# Autodesk Inventor assembly: Assembly
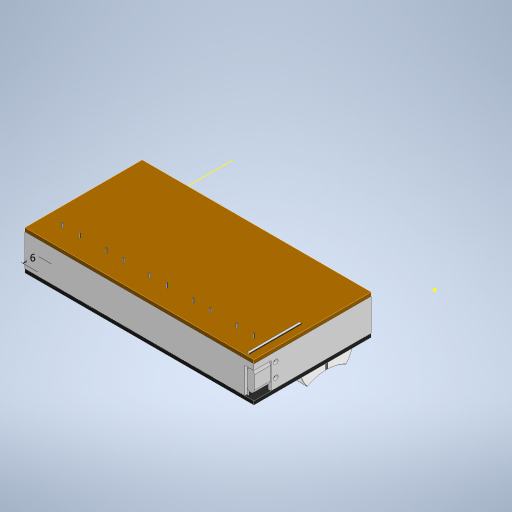
[picture p0: Inventor's stored thumbnail of the model, 512x512]
Saved by Autodesk Inventor 2023 (Build 270158000, 158)
## iProperties
Created: 2024-03-19
Part Number: Assembly
Document SubType Name: Assembly
Designer: noname
Author: noname
## Documents named in this file (10)
- C:\Users\noname\Documents\GitHub\AudMix\3dModels\Assembly.iam
- C:\Users\noname\Documents\GitHub\AudMix\3dModels\Slider\SliderAssembly.iam
- C:\Users\noname\Documents\GitHub\AudMix\3dModels\TopPCB.ipt
- C:\Users\noname\Documents\GitHub\AudMix\3dModels\Part7.ipt
- C:\Users\noname\Documents\GitHub\AudMix\3dModels\0_42_oled.ipt
- C:\Users\noname\Documents\GitHub\AudMix\3dModels\rp2040.ipt
- C:\Users\noname\Documents\GitHub\AudMix\3dModels\LedStrip\144x10.iam
- C:\Users\noname\Documents\GitHub\AudMix\3dModels\Diffuser.ipt
- C:\Users\noname\Documents\GitHub\AudMix\3dModels\Front.ipt
- C:\Users\noname\Documents\GitHub\AudMix\3dModels\Case.ipt
## Components (35 placed, 9 different names)
1. TopPCB:1 — Mate:1, Flush:1, Flush:14, Mate:9, Mate:12, Mate:16, Flush:27, Mate:17, Mate:18, Mate:19, Mate:21, Mate:23, Flush:29, Flush:32, Flush:33
2. Part7:1 — Flush:15, Mate:22, Mate:25, Flush:34, Flush:35
3. rp2040:1 — Flush:32, Flush:33
4. Front:1 — Mate:22, Mate:23, Flush:29, Mate:24
5. Case:1 — Mate:25, Flush:34, Flush:35
6. SliderAssembly:1 [sub-assembly] — Mate:1, Flush:1, Mate:11, Mate:12, Flush:30
7. 0_42_oled:5 — Flush:30, Mate:24
8. 144x10:1 [sub-assembly] — Flush:28, Mate:20, Mate:21, Flush:31
9. 144x10:2 [sub-assembly] — Mate:9, Mate:11, Mate:15, Flush:31
10. Diffuser:1 — Mate:15, Mate:16, Flush:27
11. Diffuser:2 — Mate:17, Mate:18, Mate:19, Flush:28, Mate:20
12. SliderAssembly:2 [sub-assembly]
13. 0_42_oled:6
14. 144x10:3 [sub-assembly]
15. 144x10:4 [sub-assembly]
16. Diffuser:3
17. Diffuser:4
18. SliderAssembly:3 [sub-assembly]
19. 0_42_oled:7
20. 144x10:5 [sub-assembly]
21. 144x10:6 [sub-assembly]
22. Diffuser:5
23. Diffuser:6
24. SliderAssembly:4 [sub-assembly]
25. 0_42_oled:8
26. 144x10:7 [sub-assembly]
27. 144x10:8 [sub-assembly]
28. Diffuser:7
29. Diffuser:8
30. SliderAssembly:5 [sub-assembly]
31. 0_42_oled:9
32. 144x10:9 [sub-assembly]
33. 144x10:10 [sub-assembly]
34. Diffuser:9
35. Diffuser:10
## Component patterns: (5 elements, first: SliderAssembly:1 + 0_42_oled:5 + 144x10:1 + 144x10:2 + Diffuser:1 + Diffuser:2)
## Relationships (27: Mate 15, Flush 12)
- Mate:1 (7 mm): TopPCB:1 ↔ SliderAssembly:1
- Flush:1: TopPCB:1 ↔ SliderAssembly:1
- Flush:14 (14 mm): TopPCB:1
- Flush:15: Part7:1
- Mate:9: TopPCB:1 ↔ 144x10:2
- Mate:11 (3 mm): SliderAssembly:1 ↔ 144x10:2
- Mate:12 (3.5 mm): TopPCB:1 ↔ SliderAssembly:1
- Mate:15: 144x10:2 ↔ Diffuser:1
- Mate:16: TopPCB:1 ↔ Diffuser:1
- Flush:27: TopPCB:1 ↔ Diffuser:1
- Mate:17: TopPCB:1 ↔ Diffuser:2
- Mate:18: TopPCB:1 ↔ Diffuser:2
- Mate:19: TopPCB:1 ↔ Diffuser:2
- Flush:28 (-1 mm): 144x10:1 ↔ Diffuser:2
- Mate:20: 144x10:1 ↔ Diffuser:2
- Mate:21: TopPCB:1 ↔ 144x10:1
- Mate:22: Part7:1 ↔ Front:1
- Mate:23: TopPCB:1 ↔ Front:1
- Flush:29: TopPCB:1 ↔ Front:1
- Flush:30 (3.75 mm): SliderAssembly:1 ↔ 0_42_oled:5
- Mate:24 (0.5 mm): Front:1 ↔ 0_42_oled:5
- Flush:31: 144x10:1 ↔ 144x10:2
- Flush:32 (3 mm): TopPCB:1 ↔ rp2040:1
- Flush:33 (1 mm): TopPCB:1 ↔ rp2040:1
- Mate:25: Part7:1 ↔ Case:1
- Flush:34: Part7:1 ↔ Case:1
- Flush:35: Part7:1 ↔ Case:1
